# Autodesk Inventor assembly: RMDL2.0¡ª¡ª00
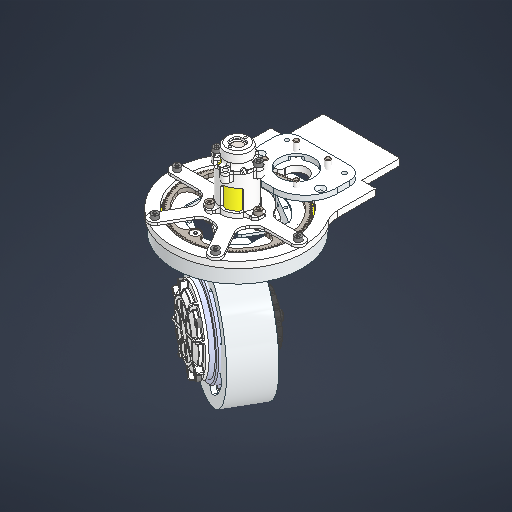
[picture p0: Inventor's stored thumbnail of the model, 512x512]
Saved by Autodesk Inventor 2025 (Build 290162000, 162)
## iProperties
Created: 2022-07-31
Part Number: RMDL2.0¡ª¡ª00
Description: STEP AP214
Document SubType Name: Assembly
Designer: XH
Sending System: SolidWorks 2021
Preprocessor: SwSTEP 2.0
Title: RMDL2.0¡ª¡ª00.STEP
Revision Number: ÈÎºÎ
## Documents named in this file (28)
- C:\1A_Engineering_files\RCInventor\铝件版本\轮系\舵轮\RMDL2.0——00.iam
- C:\1A_Engineering_files\RCInventor\铝件版本\轮系\舵轮\RMDL02¡ª¡ª0101.ipt
- C:\1A_Engineering_files\RCInventor\铝件版本\轮系\舵轮\RMDL02¡ª¡ª0102.ipt
- C:\1A_Engineering_files\RCInventor\铝件版本\轮系\舵轮\RMDL02¡ª¡ª0103.ipt
- C:\1A_Engineering_files\RCInventor\铝件版本\轮系\舵轮\61814ZZ.ipt
- C:\1A_Engineering_files\RCInventor\铝件版本\轮系\舵轮\ÄÚ¾¶5  12Â·2A»¬»·.ipt
- C:\1A_Engineering_files\RCInventor\铝件版本\轮系\舵轮\±àÂëÆ÷´ÅÌú.ipt
- C:\1A_Engineering_files\RCInventor\铝件版本\轮系\舵轮\M3×ÔÄ¥ÂÁÖù.ipt
- C:\1A_Engineering_files\RCInventor\铝件版本\轮系\舵轮\RMDL02¡ª¡ª0201.ipt
- C:\1A_Engineering_files\RCInventor\铝件版本\轮系\舵轮\RMDL02Ô²Öù³ÝÂÖ136¡Á0.6.ipt
- C:\1A_Engineering_files\RCInventor\铝件版本\轮系\舵轮\RMDL02¡ª¡ª0202.ipt
- C:\1A_Engineering_files\RCInventor\铝件版本\轮系\舵轮\RMDL02¡ª¡ª0301.ipt
- C:\1A_Engineering_files\RCInventor\铝件版本\轮系\舵轮\RMDL02¡ª¡ª0302.ipt
- C:\1A_Engineering_files\RCInventor\铝件版本\轮系\舵轮\RMDL02¡ª¡ª0401.ipt
- C:\1A_Engineering_files\RCInventor\铝件版本\轮系\舵轮\RMDL02¡ª¡ª0402.ipt
- C:\1A_Engineering_files\RCInventor\铝件版本\轮系\舵轮\RMDL02¡ª¡ª0404.ipt
- C:\1A_Engineering_files\RCInventor\铝件版本\轮系\舵轮\RMDL02¡ª¡ª0403.ipt
- C:\1A_Engineering_files\RCInventor\铝件版本\轮系\舵轮\RMDL02¡ª¡ª0405.ipt
- C:\1A_Engineering_files\RCInventor\铝件版本\轮系\舵轮\GB£¯T70£®3-2000ÄÚÁù½Ç³ÁÍ·ÂÝ¶¤M3¡Á8.ipt
- C:\1A_Engineering_files\RCInventor\铝件版本\轮系\舵轮\GB£¯T70£®2-2000ÄÚÁù½ÇÆ½Ô²Í·ÂÝ¶¤M4¡Á8.ipt
- C:\1A_Engineering_files\RCInventor\铝件版本\轮系\舵轮\GB£¯T70£®3-2000ÄÚÁù½Ç³ÁÍ·ÂÝ¶¤M3¡Á10.ipt
- C:\1A_Engineering_files\RCInventor\铝件版本\轮系\舵轮\ÄÚÁù½ÇÔ²ÖùÍ· ×Ô¹¥ÂÝ¶¤M3¡Á10.ipt
- C:\1A_Engineering_files\RCInventor\铝件版本\轮系\舵轮\ÄÚÁù½ÇÔ²ÖùÍ· ×Ô¹¥ÂÝ¶¤M3¡Á6.ipt
- C:\1A_Engineering_files\RCInventor\铝件版本\轮系\舵轮\GB£¯T70£®1-2000ÄÚÁù½ÇÔ²ÖùÍ·ÂÝ¶¤M3¡Á12.ipt
- C:\1A_Engineering_files\RCInventor\铝件版本\轮系\舵轮\GB£¯T70£®2-2000ÄÚÁù½ÇÆ½Ô²Í·ÂÝ¶¤M4¡Á6.ipt
- C:\1A_Engineering_files\RCInventor\铝件版本\轮系\舵轮\GB£¯T70£®2-2000ÄÚÁù½ÇÆ½Ô²Í·ÂÝ¶¤M3¡Á6.ipt
- C:\1A_Engineering_files\RCInventor\铝件版本\轮系\舵轮\¶æÂÖÂÖì±100mm.ipt
- C:\1A_Engineering_files\RCInventor\铝件版本\轮系\¿Í»§Ä£ÐÍ M3508¼õËÙÏä ¼õ±È268£º17.0004.ipt
## Components (38 placed, 38 different names)
1. RMDL02¡ª¡ª0101_1 — 配合:3, 配合:4, 配合:5, 配合:6, 配合:7
2. RMDL02¡ª¡ª0102_2 — 配合:8, 配合:9
3. RMDL02¡ª¡ª0103_3
4. 61814ZZ_9 — 配合:3, 配合:4, 配合:8, 配合:9
5. ÄÚ¾¶5  12Â·2A»¬»·_11
6. ±àÂëÆ÷´ÅÌú_12
7. M3×ÔÄ¥ÂÁÖù_13 — 配合:11
8. RMDL02¡ª¡ª0201_30
9. RMDL02Ô²Öù³ÝÂÖ136¡Á0.6_31
10. RMDL02¡ª¡ª0202_34 — 配合:5, 配合:6, 配合:7, 配合:10
11. RMDL02¡ª¡ª0301_37
12. RMDL02¡ª¡ª0302_38
13. RMDL02¡ª¡ª0401_43
14. RMDL02¡ª¡ª0402_44
15. RMDL02¡ª¡ª0404_45
16. RMDL02¡ª¡ª0403_46
17. RMDL02¡ª¡ª0405_47 — 配合:10, 配合:11
18. GB£¯T70£®3-2000ÄÚÁù½Ç³ÁÍ·ÂÝ¶¤M3¡Á8_49
19. GB£¯T70£®2-2000ÄÚÁù½ÇÆ½Ô²Í·ÂÝ¶¤M4¡Á8_50
20. GB£¯T70£®2-2000ÄÚÁù½ÇÆ½Ô²Í·ÂÝ¶¤M4¡Á8_51
21. GB£¯T70£®3-2000ÄÚÁù½Ç³ÁÍ·ÂÝ¶¤M3¡Á10_52
22. GB£¯T70£®3-2000ÄÚÁù½Ç³ÁÍ·ÂÝ¶¤M3¡Á10_53
23. GB£¯T70£®3-2000ÄÚÁù½Ç³ÁÍ·ÂÝ¶¤M3¡Á10_54
24. GB£¯T70£®3-2000ÄÚÁù½Ç³ÁÍ·ÂÝ¶¤M3¡Á10_55
25. ÄÚÁù½ÇÔ²ÖùÍ· ×Ô¹¥ÂÝ¶¤M3¡Á10_63
26. ÄÚÁù½ÇÔ²ÖùÍ· ×Ô¹¥ÂÝ¶¤M3¡Á10_64
27. ÄÚÁù½ÇÔ²ÖùÍ· ×Ô¹¥ÂÝ¶¤M3¡Á10_65
28. ÄÚÁù½ÇÔ²ÖùÍ· ×Ô¹¥ÂÝ¶¤M3¡Á6_66
29. ÄÚÁù½ÇÔ²ÖùÍ· ×Ô¹¥ÂÝ¶¤M3¡Á6_67
30. GB£¯T70£®1-2000ÄÚÁù½ÇÔ²ÖùÍ·ÂÝ¶¤M3¡Á12_68
31. GB£¯T70£®1-2000ÄÚÁù½ÇÔ²ÖùÍ·ÂÝ¶¤M3¡Á12_69
32. GB£¯T70£®1-2000ÄÚÁù½ÇÔ²ÖùÍ·ÂÝ¶¤M3¡Á12_70
33. GB£¯T70£®1-2000ÄÚÁù½ÇÔ²ÖùÍ·ÂÝ¶¤M3¡Á12_71
34. GB£¯T70£®2-2000ÄÚÁù½ÇÆ½Ô²Í·ÂÝ¶¤M4¡Á8_72
35. GB£¯T70£®2-2000ÄÚÁù½ÇÆ½Ô²Í·ÂÝ¶¤M4¡Á6_73
36. GB£¯T70£®2-2000ÄÚÁù½ÇÆ½Ô²Í·ÂÝ¶¤M3¡Á6_85
37. ¶æÂÖÂÖì±100mm:1 — 配合:1, 配合:2
38. ¿Í»§Ä£ÐÍ M3508¼õËÙÏä ¼õ±È268£º17.0004:1 — 配合:1, 配合:2
## Relationships (11: Mate 11)
- 配合:1 [Mate]: ¶æÂÖÂÖì±100mm:1 ↔ ¿Í»§Ä£ÐÍ M3508¼õËÙÏä ¼õ±È268£º17.0004:1
- 配合:2 [Mate]: ¶æÂÖÂÖì±100mm:1 ↔ ¿Í»§Ä£ÐÍ M3508¼õËÙÏä ¼õ±È268£º17.0004:1
- 配合:3 [Mate]: RMDL02¡ª¡ª0101_1 ↔ 61814ZZ_9
- 配合:4 [Mate]: RMDL02¡ª¡ª0101_1 ↔ 61814ZZ_9
- 配合:5 [Mate]: RMDL02¡ª¡ª0101_1 ↔ RMDL02¡ª¡ª0202_34
- 配合:6 [Mate]: RMDL02¡ª¡ª0101_1 ↔ RMDL02¡ª¡ª0202_34
- 配合:7 [Mate]: RMDL02¡ª¡ª0101_1 ↔ RMDL02¡ª¡ª0202_34
- 配合:8 [Mate]: RMDL02¡ª¡ª0102_2 ↔ 61814ZZ_9
- 配合:9 [Mate]: RMDL02¡ª¡ª0102_2 ↔ 61814ZZ_9
- 配合:10 [Mate]: RMDL02¡ª¡ª0202_34 ↔ RMDL02¡ª¡ª0405_47
- 配合:11 [Mate]: M3×ÔÄ¥ÂÁÖù_13 ↔ RMDL02¡ª¡ª0405_47
